# Autodesk Inventor assembly: F_TOPO
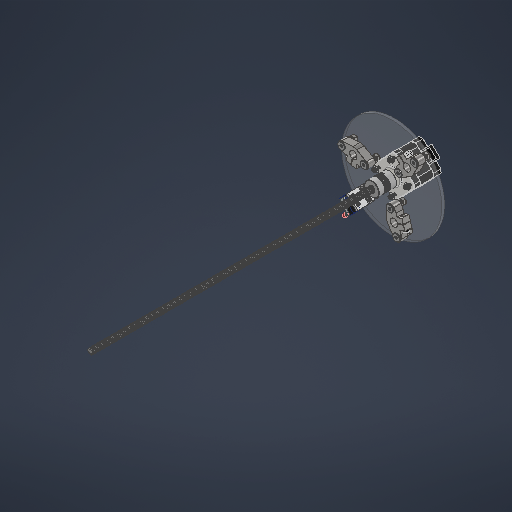
[picture p0: Inventor's stored thumbnail of the model, 512x512]
Saved by Autodesk Inventor 2025.2 (Build 292293000, 293)
## iProperties
Created: 2025-05-02
Part Number: F_TOPO
Document SubType Name: Assembly
Designer: Nelson
Author: Nelson
## Documents named in this file (20)
- C:\Users\Tiago\Documents\Inventor\Exp. Braço v1\F_TOPO.iam
- C:\Users\Tiago\Documents\Inventor\Exp. Braço v1\Topo.ipt
- C:\Users\Tiago\Documents\Inventor\Exp. Braço v1\Lead screw 2pitch_8lead_400mm.ipt
- C:\Users\Tiago\Documents\Inventor\Exp. Braço v1\NEMA17 42-38.ipt
- C:\Users\Tiago\Documents\Inventor\Exp. Braço v1\shaft_coupler 5mm_to_8mm.ipt
- C:\Users\Tiago\Documents\Inventor\Exp. Braço v1\Linear_Shaft_Support_SHF10.ipt
- C:\Users\Tiago\Documents\Inventor\Exp. Braço v1\Anilha_M3.ipt
- C:\Users\Tiago\Documents\Inventor\Exp. Braço v1\M3 x0.5 ALT (...).ipt
- C:\Users\Tiago\Documents\Inventor\Exp. Braço v1\Porca_sextavada(3M).ipt
- C:\Users\Tiago\Documents\Inventor\Exp. Braço v1\M3 x8L_hexagonal_BigHEAD.ipt
- C:\Users\Tiago\Documents\Inventor\Exp. Braço v1\M5x16L_Hex.ipt
- C:\Users\Tiago\Documents\Inventor\Exp. Braço v1\M5_nylonLock_Nut.ipt
- C:\Users\Tiago\Documents\Inventor\Exp. Braço v1\M5x20L_Hex.ipt
- C:\Users\Tiago\Documents\Inventor\Exp. Braço v1\LimitSwitch_TopHolder.ipt
- C:\Users\Tiago\Documents\Inventor\Exp. Braço v1\Limit switch\complete limit switch\complete limit switch\complete limit switch.ipt
- C:\Users\Tiago\Documents\Inventor\Exp. Braço v1\M2x12L_Hex.ipt
- M2x12L_Hex.ipt
- C:\Users\Tiago\Documents\Inventor\Exp. Braço v1\Porca_sextavada(M2).ipt
- C:\Users\Tiago\Documents\Inventor\Exp. Braço v1\M5 x12L_Hex_C.ipt
- M5 x12L_Hex_C.ipt
## Components (40 placed, 17 different names)
1. Topo:1 — Mate:1, Mate:2, Mate:3, Mate:4, Mate:5, Mate:6, Mate:7, Mate:8, Mate:9, Mate:10, Mate:11, Mate:12, Insert:6, Mate:22, Mate:23, Mate:24, Insert:11, Insert:12, Insert:13, Insert:24, Insert:26, Insert:27, Insert:28, Insert:29, Insert:30, Mate:25, Mate:26, Mate:30
2. Lead screw 2pitch_8lead_400mm:1 — Mate:13, Mate:14, Mate:16, Rotation:1
3. NEMA17 42-38:1 — Mate:2, Mate:3, Mate:14, Mate:15, Mate:16, Mate:24, Angle:1
4. shaft_coupler 5mm_to_8mm:1 — Mate:13, Mate:15, Rotation:1
5. Linear_Shaft_Support_SHF10:1 — Mate:4, Mate:9, Mate:10, Insert:20, Insert:21, Insert:39
6. Linear_Shaft_Support_SHF10:2 — Mate:5, Mate:7, Mate:12, Insert:18, Insert:19, Insert:40
7. Linear_Shaft_Support_SHF10:3 — Mate:6, Mate:8, Mate:11, Insert:23, Insert:31, Insert:38
8. Anilha_M3:1 — Insert:11, Insert:17
9. Anilha_M3:2 — Insert:12, Insert:16
10. Anilha_M3:3 — Insert:6, Insert:14
11. Anilha_M3:4 — Insert:13, Insert:15
12. M3 x0.5 ALT (...):5 — Mate:20, Insert:32
13. M3 x0.5 ALT (...):6 — Mate:21, Insert:33
14. Porca_sextavada(3M):1 — Mate:21, Mate:22
15. Porca_sextavada(3M):2 — Mate:20, Mate:23
16. M3 x8L_hexagonal_BigHEAD:1 — Insert:14
17. M3 x8L_hexagonal_BigHEAD:2 — Insert:15
18. M3 x8L_hexagonal_BigHEAD:3 — Insert:16
19. M3 x8L_hexagonal_BigHEAD:4 — Insert:17
20. M5x16L_Hex:1 — Insert:18
21. M5x16L_Hex:2 — Insert:21
22. M5x16L_Hex:3 — Insert:19
23. M5x16L_Hex:4 — Insert:20
24. M5x16L_Hex:6 — Insert:23
25. M5_nylonLock_Nut:1 — Insert:24
26. M5_nylonLock_Nut:2 — Insert:30, Angle:1
27. M5_nylonLock_Nut:3 — Insert:26
28. M5_nylonLock_Nut:4 — Insert:27
29. M5_nylonLock_Nut:5 — Insert:28
30. M5_nylonLock_Nut:6 — Insert:29
31. M5x20L_Hex:1 — Insert:31
32. LimitSwitch_TopHolder:1 — Mate:25, Mate:26, Mate:27, Mate:28, Mate:29, Mate:30, Insert:32, Insert:33, Insert:36, Insert:37
33. complete limit switch:1 — Mate:27, Mate:28, Mate:29, Insert:34, Insert:35
34. M2x12L_Hex:1 — Insert:35
35. M2x12L_Hex:2 — Insert:34
36. Porca_sextavada(M2):1 — Insert:36
37. Porca_sextavada(M2):2 — Insert:37
38. M5 x12L_Hex_C:1 — Insert:38
39. M5 x12L_Hex_C:2 — Insert:39
40. M5 x12L_Hex_C:3 — Insert:40
## Relationships (58: Insert 29, Mate 27, RelateRotation 1, Angle 1)
- Mate:1: Topo:1
- Mate:2: Topo:1 ↔ NEMA17 42-38:1
- Mate:3: Topo:1 ↔ NEMA17 42-38:1
- Mate:4: Topo:1 ↔ Linear_Shaft_Support_SHF10:1
- Mate:5: Topo:1 ↔ Linear_Shaft_Support_SHF10:2
- Mate:6: Topo:1 ↔ Linear_Shaft_Support_SHF10:3
- Mate:7: Topo:1 ↔ Linear_Shaft_Support_SHF10:2
- Mate:8: Topo:1 ↔ Linear_Shaft_Support_SHF10:3
- Mate:9: Topo:1 ↔ Linear_Shaft_Support_SHF10:1
- Mate:10: Topo:1 ↔ Linear_Shaft_Support_SHF10:1
- Mate:11: Topo:1 ↔ Linear_Shaft_Support_SHF10:3
- Mate:12: Topo:1 ↔ Linear_Shaft_Support_SHF10:2
- Mate:13: Lead screw 2pitch_8lead_400mm:1 ↔ shaft_coupler 5mm_to_8mm:1
- Mate:14: Lead screw 2pitch_8lead_400mm:1 ↔ NEMA17 42-38:1
- Mate:15 (5 mm): NEMA17 42-38:1 ↔ shaft_coupler 5mm_to_8mm:1
- Mate:16 (1 mm): Lead screw 2pitch_8lead_400mm:1 ↔ NEMA17 42-38:1
- Rotation:1 [RelateRotation] (1 ul): Lead screw 2pitch_8lead_400mm:1 ↔ shaft_coupler 5mm_to_8mm:1
- Insert:6: Topo:1 ↔ Anilha_M3:3
- Mate:20: M3 x0.5 ALT (...):5 ↔ Porca_sextavada(3M):2
- Mate:21: M3 x0.5 ALT (...):6 ↔ Porca_sextavada(3M):1
- Mate:22: Topo:1 ↔ Porca_sextavada(3M):1
- Mate:23: Topo:1 ↔ Porca_sextavada(3M):2
- Mate:24 (0.044 mm): Topo:1 ↔ NEMA17 42-38:1
- Insert:11: Topo:1 ↔ Anilha_M3:1
- Insert:12: Topo:1 ↔ Anilha_M3:2
- Insert:13: Topo:1 ↔ Anilha_M3:4
- Insert:14: Anilha_M3:3 ↔ M3 x8L_hexagonal_BigHEAD:1
- Insert:15: Anilha_M3:4 ↔ M3 x8L_hexagonal_BigHEAD:2
- Insert:16: Anilha_M3:2 ↔ M3 x8L_hexagonal_BigHEAD:3
- Insert:17: Anilha_M3:1 ↔ M3 x8L_hexagonal_BigHEAD:4
- Insert:18: Linear_Shaft_Support_SHF10:2 ↔ M5x16L_Hex:1
- Insert:19: Linear_Shaft_Support_SHF10:2 ↔ M5x16L_Hex:3
- Insert:20: Linear_Shaft_Support_SHF10:1 ↔ M5x16L_Hex:4
- Insert:21: Linear_Shaft_Support_SHF10:1 ↔ M5x16L_Hex:2
- Insert:23: Linear_Shaft_Support_SHF10:3 ↔ M5x16L_Hex:6
- Insert:24: Topo:1 ↔ M5_nylonLock_Nut:1
- Insert:26: Topo:1 ↔ M5_nylonLock_Nut:3
- Insert:27: Topo:1 ↔ M5_nylonLock_Nut:4
- Insert:28: Topo:1 ↔ M5_nylonLock_Nut:5
- Insert:29: Topo:1 ↔ M5_nylonLock_Nut:6
- Insert:30: Topo:1 ↔ M5_nylonLock_Nut:2
- Angle:1 (180 deg): NEMA17 42-38:1 ↔ M5_nylonLock_Nut:2
- Insert:31: Linear_Shaft_Support_SHF10:3 ↔ M5x20L_Hex:1
- Mate:25: Topo:1 ↔ LimitSwitch_TopHolder:1
- Mate:26: Topo:1 ↔ LimitSwitch_TopHolder:1
- Mate:27: LimitSwitch_TopHolder:1 ↔ complete limit switch:1
- Mate:28: LimitSwitch_TopHolder:1 ↔ complete limit switch:1
- Mate:29: LimitSwitch_TopHolder:1 ↔ complete limit switch:1
- Mate:30: Topo:1 ↔ LimitSwitch_TopHolder:1
- Insert:32: M3 x0.5 ALT (...):5 ↔ LimitSwitch_TopHolder:1
- Insert:33: M3 x0.5 ALT (...):6 ↔ LimitSwitch_TopHolder:1
- Insert:34: complete limit switch:1 ↔ M2x12L_Hex:2
- Insert:35: complete limit switch:1 ↔ M2x12L_Hex:1
- Insert:36: LimitSwitch_TopHolder:1 ↔ Porca_sextavada(M2):1
- Insert:37: LimitSwitch_TopHolder:1 ↔ Porca_sextavada(M2):2
- Insert:38: Linear_Shaft_Support_SHF10:3 ↔ M5 x12L_Hex_C:1
- Insert:39: Linear_Shaft_Support_SHF10:1 ↔ M5 x12L_Hex_C:2
- Insert:40: Linear_Shaft_Support_SHF10:2 ↔ M5 x12L_Hex_C:3
